# Autodesk Inventor assembly: Right Hook Encoder Assembly
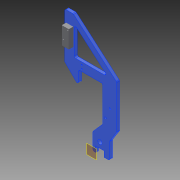
[picture p0: Inventor's stored thumbnail of the model, 180x180]
Saved by Autodesk Inventor 2013 (Build 170138000, 138)
## iProperties
Created: 2013-03-16
Part Number: Right Hook Encoder Assembly
Document SubType Name: Assembly
Designer: Arpan
Author: Arpan
## Documents named in this file (3)
- C:\Users\Arpan\Documents\GitHub\frc2013CAD\Midwest Climber\Right Hook Encoder Assembly.iam
- C:\Users\Arpan\Documents\GitHub\frc2013CAD\Midwest Climber\Limit Switch.ipt
- C:\Users\Arpan\Documents\GitHub\frc2013CAD\Midwest Climber\Bent Right Hook.ipt
## Components (2 placed, 2 different names)
1. Limit Switch:1 — Mate:1, Mate:2, Angle:1
2. Bent Right Hook:1 — Mate:1, Mate:2, Angle:1
## Relationships (3: Mate 2, Angle 1)
- Mate:1: Limit Switch:1 ↔ Bent Right Hook:1
- Mate:2: Limit Switch:1 ↔ Bent Right Hook:1
- Angle:1 (0 deg): Limit Switch:1 ↔ Bent Right Hook:1
